# Autodesk Inventor assembly: 조립_v2
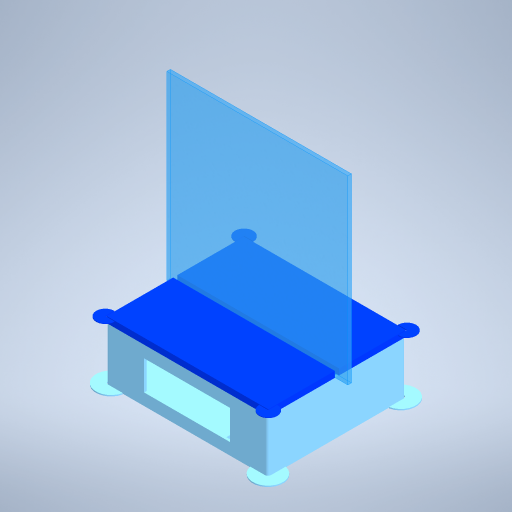
[picture p0: Inventor's stored thumbnail of the model, 512x512]
Saved by Autodesk Inventor 2023 (Build 270158000, 158)
## iProperties
Created: 2022-10-09
Part Number: 조립_v2
Document SubType Name: Assembly
Designer: 전상현
Author: 전상현
## Documents named in this file (4)
- C:\Users\전상현\Documents\Inventor\lecture\moodlight\조립_v2.iam
- C:\Users\전상현\Documents\Inventor\lecture\moodlight\case_cover_v2.ipt
- C:\Users\전상현\Documents\Inventor\lecture\moodlight\case_under_v2.ipt
- C:\Users\전상현\Documents\Inventor\lecture\moodlight\아크릴.ipt
## Components (3 placed, 3 different names)
1. case_cover_v2:1 — 메이트:3, 메이트:4, 플러쉬:2, 메이트:6, 메이트:7
2. case_under_v2:1 — 메이트:1, 메이트:2, 플러쉬:1, 메이트:3, 메이트:4, 플러쉬:2
3. 아크릴:1 — 메이트:6, 메이트:7
## Relationships (8: Mate 6, Flush 2)
- 메이트:1 [Mate]: case_under_v2:1
- 메이트:2 [Mate]: case_under_v2:1
- 플러쉬:1 [Flush]: case_under_v2:1
- 메이트:3 [Mate]: case_cover_v2:1 ↔ case_under_v2:1
- 메이트:4 [Mate]: case_cover_v2:1 ↔ case_under_v2:1
- 플러쉬:2 [Flush]: case_cover_v2:1 ↔ case_under_v2:1
- 메이트:6 [Mate]: case_cover_v2:1 ↔ 아크릴:1
- 메이트:7 [Mate] (0.2 mm): case_cover_v2:1 ↔ 아크릴:1
